# Autodesk Inventor assembly: Pendolo_Inverso
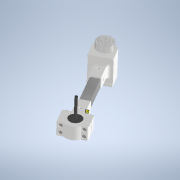
[picture p0: Inventor's stored thumbnail of the model, 180x180]
Saved by Autodesk Inventor 2020.2 (Build 242310000, 310)
## iProperties
Created: 2019-11-10
Part Number: Pendolo_Inverso
Document SubType Name: Assembly
Designer: socci
Author: socci
## Documents named in this file (14)
- C:\Users\socci\Desktop\mv-Project\04_PartDraw\Assieme_Barra2.iam
- C:\Users\socci\Documents\Inventor\Content Center Files\R2020\it-IT\Bearing GB_T 5800-2003\Rolling bearing GB_T 5800-2003 -635.ipt
- C:\Users\socci\Desktop\mv-Project\04_PartDraw\Componenti\1_Asse_cuscinetti.ipt
- C:\Users\socci\Desktop\mv-Project\04_PartDraw\Componenti\2_Connettore_inf_sup.ipt
- C:\Users\socci\Desktop\mv-Project\04_PartDraw\Componenti\3_Connettore_inf_INF.ipt
- C:\Users\socci\Desktop\mv-Project\04_PartDraw\Componenti\10_MPU_6050.ipt
- C:\Users\socci\Desktop\mv-Project\04_PartDraw\Componenti\4_barra.ipt
- C:\Users\socci\Desktop\mv-Project\04_PartDraw\Componenti\30_Connettore_sup.ipt
- C:\Users\socci\Desktop\mv-Project\04_PartDraw\Componenti\29_Motore_6mm.ipt
- C:\Users\socci\Desktop\mv-Project\04_PartDraw\Componenti\0_Sistemariferimento.ipt
- C:\Users\socci\Documents\Inventor\Content Center Files\R2020\it-IT\UNI 5739\UNI 5739 - M5 x 40.ipt
- C:\Users\socci\Documents\Inventor\Content Center Files\R2020\it-IT\IS 2016  A\IS 2016 - A5,5.ipt
- C:\Users\socci\Documents\Inventor\Content Center Files\R2020\it-IT\AS 1112 (4)\AS 1112 - M5(2).ipt
- C:\Users\socci\Documents\Inventor\Content Center Files\R2020\it-IT\AS 1110\AS 1110 - M3 x 12.ipt
## Components (31 placed, 13 different names)
1. Bearing GB/T 5800-2003 635:1 — Inserimento:3
2. 1_Asse_cuscinetti:1 — Inserimento:3, Inserimento:5, Inserimento:6
3. 2_Connettore_inf_sup:1 — Inserimento:6, Coincidente:1, Coincidente:5, Coincidente:6, Coincidente:7, Inserimento:337, Inserimento:338, Inserimento:341, Inserimento:342, Inserimento:345, Inserimento:346, Inserimento:349, Inserimento:350
4. 3_Connettore_inf_INF:1 — Inserimento:5, Coincidente:1, Inserimento:343, Inserimento:347, Inserimento:351, Inserimento:339
5. 10_MPU_6050:1
6. 4_barra:1 — Coincidente:5, Coincidente:6, Coincidente:7, Coincidente:19, Coincidente:20, Coincidente:21
7. 30_Connettore_sup:1 — Coincidente:19, Coincidente:20, Coincidente:21, Inserimento:318, Inserimento:319, Allineato:9, Coincidente:30, Coincidente:32, Inserimento:360, Inserimento:361, Inserimento:362
8. 29_Motore_6mm:1 — Inserimento:318, Inserimento:319
9. 0_Sistemariferimento:1
10. 0_Sistemariferimento:2 — Allineato:9, Coincidente:30, Coincidente:31, Allineato:10, Allineato:11
11. 0_Sistemariferimento:3 — Coincidente:31, Allineato:10, Allineato:11
12. UNI 5739 M5 x 40:8
13. IS 2016 A A5,5:15 — Inserimento:338
14. IS 2016 A A5,5:16 — Inserimento:337
15. AS 1112 (4) - Metrico M5:5 — Inserimento:339
16. UNI 5739 M5 x 40:9
17. IS 2016 A A5,5:17 — Inserimento:342
18. IS 2016 A A5,5:18 — Inserimento:341
19. AS 1112 (4) - Metrico M5:6 — Inserimento:343
20. UNI 5739 M5 x 40:10
21. IS 2016 A A5,5:19 — Inserimento:346
22. IS 2016 A A5,5:20 — Inserimento:345
23. AS 1112 (4) - Metrico M5:7 — Inserimento:347
24. UNI 5739 M5 x 40:11
25. IS 2016 A A5,5:21 — Inserimento:350
26. IS 2016 A A5,5:22 — Inserimento:349
27. AS 1112 (4) - Metrico M5:8 — Inserimento:351
28. AS 1110 - Metrico M3 x 12:1 — Coincidente:32
29. AS 1110 - Metrico M3 x 12:2 — Inserimento:362
30. AS 1110 - Metrico M3 x 12:3 — Inserimento:360
31. AS 1110 - Metrico M3 x 12:4 — Inserimento:361
## Relationships (37: Insert 24, Mate 10, Flush 3)
- Inserimento:3 (1.5 mm): Bearing GB/T 5800-2003 635:1 ↔ 1_Asse_cuscinetti:1
- Inserimento:5: 1_Asse_cuscinetti:1 ↔ 3_Connettore_inf_INF:1
- Inserimento:6: 1_Asse_cuscinetti:1 ↔ 2_Connettore_inf_sup:1
- Coincidente:1 [Mate] (1 mm): 2_Connettore_inf_sup:1 ↔ 3_Connettore_inf_INF:1
- Coincidente:5 [Mate] (0.5 mm): 2_Connettore_inf_sup:1 ↔ 4_barra:1
- Coincidente:6 [Mate] (0.5 mm): 2_Connettore_inf_sup:1 ↔ 4_barra:1
- Coincidente:7 [Mate]: 2_Connettore_inf_sup:1 ↔ 4_barra:1
- Coincidente:19 [Mate]: 4_barra:1 ↔ 30_Connettore_sup:1
- Coincidente:20 [Mate]: 4_barra:1 ↔ 30_Connettore_sup:1
- Coincidente:21 [Mate]: 4_barra:1 ↔ 30_Connettore_sup:1
- Inserimento:318: 30_Connettore_sup:1 ↔ 29_Motore_6mm:1
- Inserimento:319: 30_Connettore_sup:1 ↔ 29_Motore_6mm:1
- [Insert]: UNI 5739 M5 x 40:8 ↔ IS 2016 A A5,5:16
- Inserimento:337: 2_Connettore_inf_sup:1 ↔ IS 2016 A A5,5:16
- Inserimento:338: 2_Connettore_inf_sup:1 ↔ IS 2016 A A5,5:15
- Inserimento:339: 3_Connettore_inf_INF:1 ↔ AS 1112 (4) - Metrico M5:5
- [Insert]: UNI 5739 M5 x 40:9 ↔ IS 2016 A A5,5:18
- Inserimento:341: 2_Connettore_inf_sup:1 ↔ IS 2016 A A5,5:18
- Inserimento:342: 2_Connettore_inf_sup:1 ↔ IS 2016 A A5,5:17
- Inserimento:343: 3_Connettore_inf_INF:1 ↔ AS 1112 (4) - Metrico M5:6
- [Insert]: UNI 5739 M5 x 40:10 ↔ IS 2016 A A5,5:20
- Inserimento:345: 2_Connettore_inf_sup:1 ↔ IS 2016 A A5,5:20
- Inserimento:346: 2_Connettore_inf_sup:1 ↔ IS 2016 A A5,5:19
- Inserimento:347: 3_Connettore_inf_INF:1 ↔ AS 1112 (4) - Metrico M5:7
- [Insert]: UNI 5739 M5 x 40:11 ↔ IS 2016 A A5,5:22
- Inserimento:349: 2_Connettore_inf_sup:1 ↔ IS 2016 A A5,5:22
- Inserimento:350: 2_Connettore_inf_sup:1 ↔ IS 2016 A A5,5:21
- Inserimento:351: 3_Connettore_inf_INF:1 ↔ AS 1112 (4) - Metrico M5:8
- Allineato:9 [Flush] (71.45 mm): 30_Connettore_sup:1 ↔ 0_Sistemariferimento:2
- Coincidente:30 [Mate] (71.8 mm): 30_Connettore_sup:1 ↔ 0_Sistemariferimento:2
- Coincidente:31 [Mate]: 0_Sistemariferimento:2 ↔ 0_Sistemariferimento:3
- Allineato:10 [Flush]: 0_Sistemariferimento:2 ↔ 0_Sistemariferimento:3
- Allineato:11 [Flush] (-192 mm): 0_Sistemariferimento:2 ↔ 0_Sistemariferimento:3
- Coincidente:32 [Mate]: 30_Connettore_sup:1 ↔ AS 1110 - Metrico M3 x 12:1
- Inserimento:360: 30_Connettore_sup:1 ↔ AS 1110 - Metrico M3 x 12:3
- Inserimento:361: 30_Connettore_sup:1 ↔ AS 1110 - Metrico M3 x 12:4
- Inserimento:362: 30_Connettore_sup:1 ↔ AS 1110 - Metrico M3 x 12:2
## Named parameters: d535_d530_d518 = 0 mm, d539_d530_d518 = 0 mm, d543_d530_d518 = 0 mm, d547_d530_d518 = 0 mm
